# Autodesk Inventor assembly: Framing_For_Roof
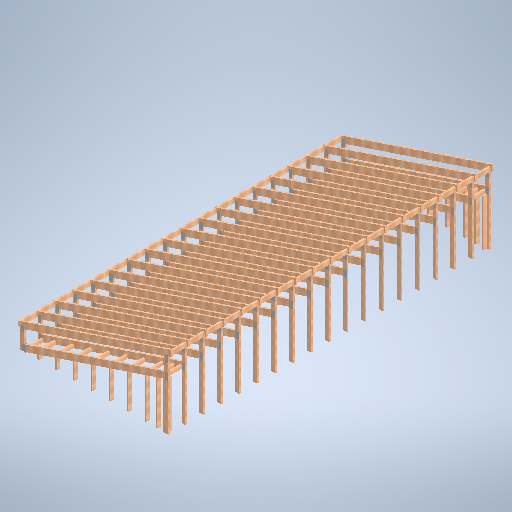
[picture p0: Inventor's stored thumbnail of the model, 512x512]
Saved by Autodesk Inventor 2025 (Build 290162010, 162A)
## iProperties
Created: 2024-10-03
Part Number: Framing_For_Roof
Document SubType Name: Assembly
Designer: Tom
Author: Tom
## Documents named in this file (17)
- C:\Users\Tom\Documents\Inventor\Mobility\Additional_Building\Framing_For_Roof.iam
- C:\Users\Tom\Documents\Inventor\Mobility\Additional_Building\Truss.iam
- C:\Users\Tom\Documents\Inventor\Mobility\Additional_Building\Stud_With_Height_4.254_Inches.ipt
- C:\Users\Tom\Documents\Inventor\Mobility\Additional_Building\Stud_With_Height_9.593_Inches.ipt
- C:\Users\Tom\Documents\Inventor\Mobility\Additional_Building\Stud_With_Height_14.931_Inches.ipt
- C:\Users\Tom\Documents\Inventor\Mobility\Additional_Building\Stud_With_Height_20.270_Inches.ipt
- C:\Users\Tom\Documents\Inventor\Mobility\Additional_Building\Stud_With_Height_25.608_Inches.ipt
- C:\Users\Tom\Documents\Inventor\Mobility\Additional_Building\Stud_With_Height_30.947_Inches.ipt
- C:\Users\Tom\Documents\Inventor\Mobility\Additional_Building\Stud_With_Height_36.285_Inches.ipt
- C:\Users\Tom\Documents\Inventor\Mobility\Additional_Building\Stud_With_Height_39.580_Inches.ipt
- C:\Users\Tom\Documents\Inventor\Mobility\Additional_Building\Stud_With_Height_41.707_Inches.ipt
- C:\Users\Tom\Documents\Inventor\Mobility\Additional_Building\Stud_With_Height_41.707_Inches_And_Cut.ipt
- C:\Users\Tom\Documents\Inventor\Mobility\Additional_Building\Subfascia_With_Dimensions_4.023_x_13.75_Inches.ipt
- C:\Users\Tom\Documents\Inventor\Mobility\Additional_Building\Subfascia_With_Dimensions_4.023_x_14.5_Inches.ipt
- C:\Users\Tom\Documents\Inventor\Mobility\Additional_Building\Subfascia_With_Dimensions_3.725_x_13.75_Inches.ipt
- C:\Users\Tom\Documents\Inventor\Mobility\Additional_Building\Subfascia_With_Dimensions_3.725_x_14.5_Inches.ipt
- C:\Users\Tom\Documents\Inventor\Mobility\Additional_Building\Support_For_Ceiling.ipt
## Components (95 placed, 16 different names)
1. Subfascia_With_Dimensions_4.023_x_13.75_Inches:1 — Mate:5, Flush:30, Flush:31
2. Subfascia_With_Dimensions_4.023_x_13.75_Inches:2 — Mate:7, Flush:35, Flush:36
3. Subfascia_With_Dimensions_3.725_x_13.75_Inches:1 — Mate:8, Flush:37, Flush:38
4. Subfascia_With_Dimensions_3.725_x_13.75_Inches:2 — Mate:10, Flush:41, Flush:42
5. Truss:1 [sub-assembly] — Mate:10, Flush:41, Flush:42
6. Truss:2 [sub-assembly] — Flush:1, Flush:2, Flush:3, Flush:4, Flush:5, Flush:6, Flush:8, Flush:9, Flush:11, Flush:12, Flush:14, Flush:15, Flush:17, Flush:18, Flush:20, Flush:21, Flush:23, Flush:24, Flush:26, Flush:27, Mate:2, Flush:28, Flush:29, Mate:3, Mate:5, Flush:30, Flush:31, Flush:32, Mate:11, Flush:44, Mate:12, Mate:13, Flush:46, Mate:14, Flush:48, Mate:15, Flush:50, Mate:16, Flush:52, Mate:17, Flush:54, Mate:18, Flush:56, Mate:19, Flush:58, Mate:20, Flush:60, Mate:21, Flush:62
7. Truss:3 [sub-assembly] — Flush:1, Flush:2, Flush:32, Mate:6, Flush:33, Flush:34, Mate:8, Flush:37, Flush:38
8. Truss:4 [sub-assembly] — Mate:9, Flush:39, Flush:40
9. Truss:5 [sub-assembly]
10. Truss:6 [sub-assembly]
11. Truss:7 [sub-assembly]
12. Truss:8 [sub-assembly]
13. Truss:9 [sub-assembly]
14. Truss:10 [sub-assembly]
15. Truss:11 [sub-assembly]
16. Truss:12 [sub-assembly]
17. Truss:13 [sub-assembly]
18. Truss:14 [sub-assembly]
19. Truss:15 [sub-assembly]
20. Truss:16 [sub-assembly]
21. Truss:17 [sub-assembly]
22. Truss:18 [sub-assembly]
23. Truss:19 [sub-assembly] — Mate:7, Flush:35, Flush:36
24. Stud_With_Height_4.254_Inches:1 — Flush:3, Flush:4, Flush:5, Flush:7, Flush:45
25. Stud_With_Height_9.593_Inches:1 — Flush:6, Flush:7, Flush:8, Flush:10, Flush:47
26. Stud_With_Height_14.931_Inches:1 — Flush:9, Flush:10, Flush:11, Flush:13, Flush:49
27. Stud_With_Height_20.270_Inches:1 — Flush:12, Flush:13, Flush:14, Flush:16, Flush:51
28. Stud_With_Height_25.608_Inches:1 — Flush:15, Flush:16, Flush:17, Flush:19, Flush:53
29. Stud_With_Height_30.947_Inches:1 — Flush:18, Flush:19, Flush:20, Flush:22, Flush:55
30. Stud_With_Height_36.285_Inches:1 — Flush:21, Flush:22, Flush:23, Flush:25, Flush:57
31. Stud_With_Height_39.580_Inches:1 — Flush:24, Flush:25, Flush:26, Flush:59
32. Stud_With_Height_41.707_Inches_And_Cut:1 — Flush:27, Mate:2, Flush:28, Mate:4, Flush:61
33. Stud_With_Height_4.254_Inches:2
34. Stud_With_Height_9.593_Inches:2
35. Stud_With_Height_14.931_Inches:2
36. Stud_With_Height_20.270_Inches:2
37. Stud_With_Height_25.608_Inches:2
38. Stud_With_Height_30.947_Inches:2
39. Stud_With_Height_36.285_Inches:2
40. Stud_With_Height_39.580_Inches:2
41. Stud_With_Height_41.707_Inches_And_Cut:2
42. Stud_With_Height_41.707_Inches:1 — Flush:29, Mate:3, Mate:4
43. Stud_With_Height_41.707_Inches:2
44. Subfascia_With_Dimensions_4.023_x_14.5_Inches:1 — Mate:6, Flush:33, Flush:34
45. Subfascia_With_Dimensions_4.023_x_14.5_Inches:2
46. Subfascia_With_Dimensions_4.023_x_14.5_Inches:3
47. Subfascia_With_Dimensions_4.023_x_14.5_Inches:4
48. Subfascia_With_Dimensions_4.023_x_14.5_Inches:5
49. Subfascia_With_Dimensions_4.023_x_14.5_Inches:6
50. Subfascia_With_Dimensions_4.023_x_14.5_Inches:7
51. Subfascia_With_Dimensions_4.023_x_14.5_Inches:8
52. Subfascia_With_Dimensions_4.023_x_14.5_Inches:9
53. Subfascia_With_Dimensions_4.023_x_14.5_Inches:10
54. Subfascia_With_Dimensions_4.023_x_14.5_Inches:11
55. Subfascia_With_Dimensions_4.023_x_14.5_Inches:12
56. Subfascia_With_Dimensions_4.023_x_14.5_Inches:13
57. Subfascia_With_Dimensions_4.023_x_14.5_Inches:14
58. Subfascia_With_Dimensions_4.023_x_14.5_Inches:15
59. Subfascia_With_Dimensions_4.023_x_14.5_Inches:16
60. Subfascia_With_Dimensions_3.725_x_14.5_Inches:1 — Mate:9, Flush:39, Flush:40
61. Subfascia_With_Dimensions_3.725_x_14.5_Inches:2
62. Subfascia_With_Dimensions_3.725_x_14.5_Inches:3
63. Subfascia_With_Dimensions_3.725_x_14.5_Inches:4
64. Subfascia_With_Dimensions_3.725_x_14.5_Inches:5
65. Subfascia_With_Dimensions_3.725_x_14.5_Inches:6
66. Subfascia_With_Dimensions_3.725_x_14.5_Inches:7
67. Subfascia_With_Dimensions_3.725_x_14.5_Inches:8
68. Subfascia_With_Dimensions_3.725_x_14.5_Inches:9
69. Subfascia_With_Dimensions_3.725_x_14.5_Inches:10
70. Subfascia_With_Dimensions_3.725_x_14.5_Inches:11
71. Subfascia_With_Dimensions_3.725_x_14.5_Inches:12
72. Subfascia_With_Dimensions_3.725_x_14.5_Inches:13
73. Subfascia_With_Dimensions_3.725_x_14.5_Inches:14
74. Subfascia_With_Dimensions_3.725_x_14.5_Inches:15
75. Subfascia_With_Dimensions_3.725_x_14.5_Inches:16
76. Support_For_Ceiling:1 — Mate:11, Flush:44, Mate:12
77. Support_For_Ceiling:2 — Mate:13, Flush:45, Flush:46
78. Support_For_Ceiling:3 — Mate:14, Flush:47, Flush:48
79. Support_For_Ceiling:4 — Mate:15, Flush:49, Flush:50
80. Support_For_Ceiling:5 — Mate:16, Flush:51, Flush:52
81. Support_For_Ceiling:6 — Mate:17, Flush:53, Flush:54
82. Support_For_Ceiling:7 — Mate:18, Flush:55, Flush:56
83. Support_For_Ceiling:8 — Mate:19, Flush:57, Flush:58
84. Support_For_Ceiling:9 — Mate:20, Flush:59, Flush:60
85. Support_For_Ceiling:10 — Mate:21, Flush:61, Flush:62
86. Support_For_Ceiling:11
87. Support_For_Ceiling:12
88. Support_For_Ceiling:13
89. Support_For_Ceiling:14
90. Support_For_Ceiling:15
91. Support_For_Ceiling:16
92. Support_For_Ceiling:17
93. Support_For_Ceiling:18
94. Support_For_Ceiling:19
95. Support_For_Ceiling:20
## Component patterns: (2 elements, first: Truss:1), (17 elements, first: Truss:3), (2 elements, first: Stud_With_Height_4.254_Inches:1 + Stud_With_Height_9.593_Inches:1 + Stud_With_Height_14.931_Inches:1 + Stud_With_Height_20.270_Inches:1 + Stud_With_Height_25.608_Inches:1 + Stud_With_Height_30.947_Inches:1 + Stud_With_Height_36.285_Inches:1 + Stud_With_Height_39.580_Inches:1 + Stud_With_Height_41.707_Inches_And_Cut:1), (2 elements, first: Stud_With_Height_41.707_Inches:1), (16 elements, first: Subfascia_With_Dimensions_4.023_x_14.5_Inches:1), (16 elements, first: Subfascia_With_Dimensions_3.725_x_14.5_Inches:1), (2 elements, first: Support_For_Ceiling:1 + Support_For_Ceiling:2 + Support_For_Ceiling:3 + Support_For_Ceiling:4 + Support_For_Ceiling:5 + Support_For_Ceiling:6 + Support_For_Ceiling:7 + Support_For_Ceiling:8 + Support_For_Ceiling:9 + Support_For_Ceiling:10)
## Relationships (81: Flush 61, Mate 20)
- Flush:1: Truss:2 ↔ Truss:3
- Flush:2: Truss:2 ↔ Truss:3
- Flush:3: Truss:2 ↔ Stud_With_Height_4.254_Inches:1
- Flush:4 (374.65 mm): Truss:2 ↔ Stud_With_Height_4.254_Inches:1
- Flush:5: Truss:2 ↔ Stud_With_Height_4.254_Inches:1
- Flush:6: Truss:2 ↔ Stud_With_Height_9.593_Inches:1
- Flush:7 (406.4 mm): Stud_With_Height_4.254_Inches:1 ↔ Stud_With_Height_9.593_Inches:1
- Flush:8: Truss:2 ↔ Stud_With_Height_9.593_Inches:1
- Flush:9: Truss:2 ↔ Stud_With_Height_14.931_Inches:1
- Flush:10 (406.4 mm): Stud_With_Height_9.593_Inches:1 ↔ Stud_With_Height_14.931_Inches:1
- Flush:11: Truss:2 ↔ Stud_With_Height_14.931_Inches:1
- Flush:12: Truss:2 ↔ Stud_With_Height_20.270_Inches:1
- Flush:13 (406.4 mm): Stud_With_Height_14.931_Inches:1 ↔ Stud_With_Height_20.270_Inches:1
- Flush:14: Truss:2 ↔ Stud_With_Height_20.270_Inches:1
- Flush:15: Truss:2 ↔ Stud_With_Height_25.608_Inches:1
- Flush:16 (406.4 mm): Stud_With_Height_20.270_Inches:1 ↔ Stud_With_Height_25.608_Inches:1
- Flush:17: Truss:2 ↔ Stud_With_Height_25.608_Inches:1
- Flush:18: Truss:2 ↔ Stud_With_Height_30.947_Inches:1
- Flush:19 (406.4 mm): Stud_With_Height_25.608_Inches:1 ↔ Stud_With_Height_30.947_Inches:1
- Flush:20: Truss:2 ↔ Stud_With_Height_30.947_Inches:1
- Flush:21: Truss:2 ↔ Stud_With_Height_36.285_Inches:1
- Flush:22 (406.4 mm): Stud_With_Height_30.947_Inches:1 ↔ Stud_With_Height_36.285_Inches:1
- Flush:23: Truss:2 ↔ Stud_With_Height_36.285_Inches:1
- Flush:24: Truss:2 ↔ Stud_With_Height_39.580_Inches:1
- Flush:25 (250.825 mm): Stud_With_Height_36.285_Inches:1 ↔ Stud_With_Height_39.580_Inches:1
- Flush:26: Truss:2 ↔ Stud_With_Height_39.580_Inches:1
- Flush:27: Truss:2 ↔ Stud_With_Height_41.707_Inches_And_Cut:1
- Mate:2: Truss:2 ↔ Stud_With_Height_41.707_Inches_And_Cut:1
- Flush:28: Truss:2 ↔ Stud_With_Height_41.707_Inches_And_Cut:1
- Flush:29: Truss:2 ↔ Stud_With_Height_41.707_Inches:1
- Mate:3: Truss:2 ↔ Stud_With_Height_41.707_Inches:1
- Mate:4: Stud_With_Height_41.707_Inches_And_Cut:1 ↔ Stud_With_Height_41.707_Inches:1
- Mate:5: Subfascia_With_Dimensions_4.023_x_13.75_Inches:1 ↔ Truss:2
- Flush:30: Subfascia_With_Dimensions_4.023_x_13.75_Inches:1 ↔ Truss:2
- Flush:31: Subfascia_With_Dimensions_4.023_x_13.75_Inches:1 ↔ Truss:2
- Flush:32 (387.35 mm): Truss:2 ↔ Truss:3
- Mate:6: Truss:3 ↔ Subfascia_With_Dimensions_4.023_x_14.5_Inches:1
- Flush:33: Truss:3 ↔ Subfascia_With_Dimensions_4.023_x_14.5_Inches:1
- Flush:34: Truss:3 ↔ Subfascia_With_Dimensions_4.023_x_14.5_Inches:1
- Mate:7: Subfascia_With_Dimensions_4.023_x_13.75_Inches:2 ↔ Truss:19
- Flush:35: Subfascia_With_Dimensions_4.023_x_13.75_Inches:2 ↔ Truss:19
- Flush:36: Subfascia_With_Dimensions_4.023_x_13.75_Inches:2 ↔ Truss:19
- Mate:8: Subfascia_With_Dimensions_3.725_x_13.75_Inches:1 ↔ Truss:3
- Flush:37: Subfascia_With_Dimensions_3.725_x_13.75_Inches:1 ↔ Truss:3
- Flush:38 (25.4 mm): Subfascia_With_Dimensions_3.725_x_13.75_Inches:1 ↔ Truss:3
- Mate:9: Truss:4 ↔ Subfascia_With_Dimensions_3.725_x_14.5_Inches:1
- Flush:39: Truss:4 ↔ Subfascia_With_Dimensions_3.725_x_14.5_Inches:1
- Flush:40 (25.4 mm): Truss:4 ↔ Subfascia_With_Dimensions_3.725_x_14.5_Inches:1
- Mate:10: Subfascia_With_Dimensions_3.725_x_13.75_Inches:2 ↔ Truss:1
- Flush:41: Subfascia_With_Dimensions_3.725_x_13.75_Inches:2 ↔ Truss:1
- Flush:42 (25.4 mm): Subfascia_With_Dimensions_3.725_x_13.75_Inches:2 ↔ Truss:1
- Mate:11: Truss:2 ↔ Support_For_Ceiling:1
- Flush:44: Truss:2 ↔ Support_For_Ceiling:1
- Mate:12: Truss:2 ↔ Support_For_Ceiling:1
- Mate:13: Truss:2 ↔ Support_For_Ceiling:2
- Flush:45: Stud_With_Height_4.254_Inches:1 ↔ Support_For_Ceiling:2
- Flush:46: Truss:2 ↔ Support_For_Ceiling:2
- Mate:14: Truss:2 ↔ Support_For_Ceiling:3
- Flush:47: Stud_With_Height_9.593_Inches:1 ↔ Support_For_Ceiling:3
- Flush:48: Truss:2 ↔ Support_For_Ceiling:3
- Mate:15: Truss:2 ↔ Support_For_Ceiling:4
- Flush:49: Stud_With_Height_14.931_Inches:1 ↔ Support_For_Ceiling:4
- Flush:50: Truss:2 ↔ Support_For_Ceiling:4
- Mate:16: Truss:2 ↔ Support_For_Ceiling:5
- Flush:51: Stud_With_Height_20.270_Inches:1 ↔ Support_For_Ceiling:5
- Flush:52: Truss:2 ↔ Support_For_Ceiling:5
- Mate:17: Truss:2 ↔ Support_For_Ceiling:6
- Flush:53: Stud_With_Height_25.608_Inches:1 ↔ Support_For_Ceiling:6
- Flush:54: Truss:2 ↔ Support_For_Ceiling:6
- Mate:18: Truss:2 ↔ Support_For_Ceiling:7
- Flush:55: Stud_With_Height_30.947_Inches:1 ↔ Support_For_Ceiling:7
- Flush:56: Truss:2 ↔ Support_For_Ceiling:7
- Mate:19: Truss:2 ↔ Support_For_Ceiling:8
- Flush:57: Stud_With_Height_36.285_Inches:1 ↔ Support_For_Ceiling:8
- Flush:58: Truss:2 ↔ Support_For_Ceiling:8
- Mate:20: Truss:2 ↔ Support_For_Ceiling:9
- Flush:59: Stud_With_Height_39.580_Inches:1 ↔ Support_For_Ceiling:9
- Flush:60: Truss:2 ↔ Support_For_Ceiling:9
- Mate:21: Truss:2 ↔ Support_For_Ceiling:10
- Flush:61: Stud_With_Height_41.707_Inches_And_Cut:1 ↔ Support_For_Ceiling:10
- Flush:62: Truss:2 ↔ Support_For_Ceiling:10
